# Autodesk Inventor assembly: ASY Beshkino_bio_tank
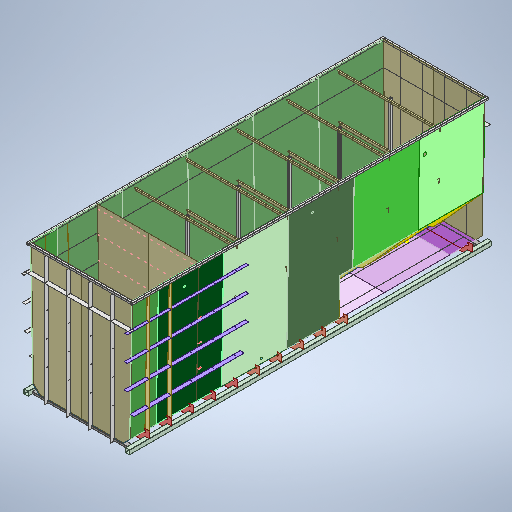
[picture p0: Inventor's stored thumbnail of the model, 512x512]
Saved by Autodesk Inventor 2025 (Build 290162010, 162A)
## iProperties
Created: 2024-07-21
Part Number: ASY Beshkino_bio_tank
Document SubType Name: Assembly
Designer: admin
Mass: 5.81287e+06 g
Surface Area: 2.77755e+06 cm^2
Volume: 3.12018e+06 cm^3
Density: 1.86299 g/cm^3
Author: admin
## Documents named in this file (39)
- C:\Users\pokla\Documents\Inventor\BSH_Beshkino_bio_tank\ASY Beshkino_bio_tank.iam
- C:\Users\pokla\Documents\Inventor\BSH_Beshkino_bio_tank\BSH 000 dim Beshkino_bio_tank.ipt
- C:\Users\pokla\Documents\Inventor\BSH_Beshkino_bio_tank\BSH 010 floor 1.ipt
- C:\Users\pokla\Documents\Inventor\BSH_Beshkino_bio_tank\BSH 021 rib 1.ipt
- C:\Users\pokla\Documents\Inventor\BSH_Beshkino_bio_tank\BSH 022 rib 2.ipt
- C:\Users\pokla\Documents\Inventor\BSH_Beshkino_bio_tank\BSH 061 tube 1.ipt
- C:\Users\pokla\Documents\Inventor\BSH_Beshkino_bio_tank\BSH 031 nose 1.ipt
- C:\Users\pokla\Documents\Inventor\BSH_Beshkino_bio_tank\BSH 032 board 2.ipt
- C:\Users\pokla\Documents\Inventor\BSH_Beshkino_bio_tank\BSH 033 board 3.ipt
- C:\Users\pokla\Documents\Inventor\BSH_Beshkino_bio_tank\BSH 041 stringer 1.ipt
- C:\Users\pokla\Documents\Inventor\BSH_Beshkino_bio_tank\BSH 039 back 9.ipt
- C:\Users\pokla\Documents\Inventor\BSH_Beshkino_bio_tank\BSH 041 stringer floor.ipt
- C:\Users\pokla\Documents\Inventor\BSH_Beshkino_bio_tank\BSH 062 tube 2.ipt
- C:\Users\pokla\Documents\Inventor\BSH_Beshkino_bio_tank\BSH 042 stringer 2.ipt
- C:\Users\pokla\Documents\Inventor\BSH_Beshkino_bio_tank\BSH 043 stringer 3.ipt
- C:\Users\pokla\Documents\Inventor\BSH_Beshkino_bio_tank\BSH 044 stringer 4.ipt
- C:\Users\pokla\Documents\Inventor\BSH_Beshkino_bio_tank\BSH 042 stringer floor.ipt
- C:\Users\pokla\Documents\Inventor\BSH_Beshkino_bio_tank\BSH 045 stringer 1.ipt
- C:\Users\pokla\Documents\Inventor\BSH_Beshkino_bio_tank\BSH 045 stringer 5.ipt
- C:\Users\pokla\Documents\Inventor\BSH_Beshkino_bio_tank\BSH 033 board cone 3.ipt
- C:\Users\pokla\Documents\Inventor\BSH_Beshkino_bio_tank\BSH 034 board cone 4.ipt
- C:\Users\pokla\Documents\Inventor\BSH_Beshkino_bio_tank\BSH 035 divider 1.ipt
- C:\Users\pokla\Documents\Inventor\BSH_Beshkino_bio_tank\BSH 036 divider 2.ipt
- C:\Users\pokla\Documents\Inventor\BSH_Beshkino_bio_tank\BSH 012 floor 2.ipt
- C:\Users\pokla\Documents\Inventor\BSH_Beshkino_bio_tank\BSH 037 cone 3.ipt
- C:\Users\pokla\Documents\Inventor\BSH_Beshkino_bio_tank\BSH 013 floor 3.ipt
- C:\Users\pokla\Documents\Inventor\BSH_Beshkino_bio_tank\BSH 015 board cone 5.ipt
- C:\Users\pokla\Documents\Inventor\BSH_Beshkino_bio_tank\BSH 038 divider.ipt
- C:\Users\pokla\Documents\Inventor\BSH_Beshkino_bio_tank\BSH 046 stringer 6.ipt
- C:\Users\pokla\Documents\Inventor\BSH_Beshkino_bio_tank\BSH 035 board cone 5.ipt
- C:\Users\pokla\Documents\Inventor\BSH_Beshkino_bio_tank\BSH 035 board .ipt
- C:\Users\pokla\Documents\Inventor\BSH_Beshkino_bio_tank\BSH 051 back 1.ipt
- C:\Users\pokla\Documents\Inventor\BSH_Beshkino_bio_tank\BSH 052 board 2.ipt
- C:\Users\pokla\Documents\Inventor\BSH_Beshkino_bio_tank\BSH 053 board 3.ipt
- C:\Users\pokla\Documents\Inventor\BSH_Beshkino_bio_tank\BSH 054 board cone 4.ipt
- C:\Users\pokla\Documents\Inventor\BSH_Beshkino_bio_tank\BSH 063 tube 3.ipt
- C:\Users\pokla\Documents\Inventor\BSH_Beshkino_bio_tank\BSH 064 tube 4.ipt
- C:\Users\pokla\Documents\Inventor\BSH_Beshkino_bio_tank\BSH 065 tube 5.ipt
- C:\Users\pokla\Documents\Inventor\BSH_Beshkino_bio_tank\BSH 023 rib 3.ipt
## Components (116 placed, 43 different names)
1. BSH 000 dim Beshkino_bio_tank.ipt:1
2. BSH 022 rib 2.ipt:1 — Rigid:27, Rigid:28, Rigid:29, Rigid:30, Rigid:74, Mate:104, Flush:26
3. BSH 061 tube 1.ipt:1 — Mate:1, Rigid:1, Mate:3, Flush:12, Mate:66, Mate:67, Mate:95, Flush:23
4. BSH 061 tube 1.ipt:2 — Mate:2, Rigid:1, Mate:4, Flush:3, Flush:4, Flush:16, Mate:65, Flush:20
5. BSH 062 tube 2.ipt:1 — Mate:19, Flush:12, Flush:16, Mate:65
6. BSH 062 tube 2.ipt:2 — Mate:68, Flush:20, Mate:95, Flush:23
7. BSH 010 floor 1.ipt:2 — Rigid:5, Rigid:83, Mate:77, Flush:18, Flush:19
8. BSH 010 floor 1.ipt:3 — Rigid:5, Rigid:82
9. BSH 010 floor 1.ipt:1 — Mate:5, Mate:6, Mate:7, Flush:4, Mate:10, Flush:5, Flush:11, Flush:17, Mate:70, Rigid:82, Mate:74
10. BSH 031 nose 1.ipt:1 — Mate:10, Flush:5, Mate:11, Rigid:11, Mate:73, Mate:108
11. BSH 033 board 3.ipt:1 — Flush:11, Mate:73, Mate:74, Rigid:104
12. BSH 031 nose 1.ipt:2 — Rigid:11, Rigid:53, Mate:69
13. BSH 021 rib 1.ipt:1 — Mate:4, Flush:3, Mate:5, Mate:6, Rigid:9, Mate:19, Rigid:74, Rigid:76, Rigid:109, Rigid:118, Rigid:122, Rigid:126
14. BSH 045 stringer 1:1
15. BSH 031 nose 1:3 — Mate:113
16. BSH 031 nose 1:4 — Rigid:53, Flush:112
17. BSH 033 board cone 3:1 — Mate:26, Rigid:57, Mate:30, Mate:80, Mate:83
18. BSH 031 nose 1:7 — Mate:26, Mate:30, Mate:84, Flush:21, Mate:94
19. BSH 031 nose 1:8 — Flush:8, Mate:40, Mate:111
20. BSH 033 board cone 3:2 — Rigid:57, Angle:1, Mate:49, Mate:50, Mate:64, Mate:71
21. BSH 043 stringer 3.ipt:1 — Rigid:29
22. BSH 042 stringer 2.ipt:1 — Rigid:28
23. BSH 041 stringer 1.ipt:1 — Rigid:27
24. BSH 041 stringer 1.ipt:2
25. BSH 042 stringer 2.ipt:2
26. BSH 043 stringer 3.ipt:2
27. BSH 044 stringer 4.ipt:2 — Rigid:71, Rigid:127, Mate:109
28. BSH 034 board cone 4:2 — Mate:84, Rigid:108, Mate:88, Mate:89, Mate:90, Mate:91
29. BSH 012 floor 2:1 — Rigid:66, Mate:42, Angle:1, Mate:49, Rigid:83, Mate:72, Mate:87
30. BSH 037 cone 3:1 — Mate:42, Mate:50, Mate:90
31. BSH 033 board 3:2 — Flush:17, Mate:69, Mate:70, Rigid:81
32. BSH 012 floor 2:2 — Rigid:66, Rigid:67, Mate:63, Mate:78, Mate:98
33. BSH 013 floor 3:1 — Rigid:67, Mate:40, Mate:81
34. BSH 039 back 9:2 — Rigid:90, Rigid:103
35. BSH 015 board cone 5:1 — Mate:71, Mate:72, Mate:85, Mate:86
36. BSH 038 divider:1 — Mate:77, Flush:18, Flush:19
37. BSH 046 stringer 6:1 — Mate:107, Mate:108, Mate:109, Rigid:128, Rigid:129, Rigid:130, Rigid:131
38. BSH 037 cone 3:2 — Mate:63, Mate:64, Mate:91
39. BSH 044 stringer 4:3 — Rigid:71, Rigid:72
40. BSH 044 stringer 4:4 — Rigid:72, Mate:112
41. BSH 022 rib 2:34 — Rigid:76, Mate:102, Flush:27, Rigid:127
42. BSH 020 rib 1:4 — Mate:66, Mate:67, Mate:68
43. BSH 022 rib 2:35 — Rigid:77
44. BSH 021 rib 1.ipt:2 — Rigid:9, Rigid:75, Rigid:77
45. BSH 037 cone 3:3 — Mate:78, Mate:80, Mate:88
46. BSH 037 cone 3:4 — Mate:81, Mate:83, Mate:89
47. BSH 035 board cone 5:1 — Rigid:107
48. BSH 035 board :1 — Rigid:90, Mate:85, Rigid:106
49. BSH 020 rib 1:5
50. BSH 020 rib 1:6
51. BSH 020 rib 1:7 — Rigid:94
52. BSH 020 rib 1:8 — Rigid:94
53. BSH 020 rib 1:9
54. BSH 020 rib 1:10
55. BSH 020 rib 1:11
56. BSH 051 back 1:1 — Rigid:103, Flush:21, Mate:96
57. BSH 052 board 2:1 — Rigid:104, Rigid:105
58. BSH 044 stringer 4.ipt:1 — Rigid:30
59. BSH 022 rib 2:33 — Rigid:75
60. BSH 053 board 3:1 — Rigid:105, Rigid:106
61. BSH 054 board cone 4:1 — Rigid:107, Rigid:108, Mate:86, Mate:87
62. BSH 041 stringer floor:1 — Rigid:109, Rigid:114
63. BSH 042 stringer floor:1 — Rigid:113
64. BSH 041 stringer floor:2 — Rigid:112, Rigid:114
65. BSH 041 stringer floor:3 — Rigid:112, Rigid:113
66. BSH 020 rib 1:12
67. BSH 041 stringer floor:4 — Rigid:118
68. BSH 042 stringer floor:2
69. BSH 041 stringer floor:5
70. BSH 041 stringer floor:6
71. BSH 041 stringer floor:7 — Rigid:122
72. BSH 042 stringer floor:3
73. BSH 041 stringer floor:8
74. BSH 041 stringer floor:9
75. BSH 041 stringer floor:10 — Rigid:126
76. BSH 042 stringer floor:4
77. BSH 041 stringer floor:11
78. BSH 041 stringer floor:12
79. BSH 064 tube 4:1 — Mate:100, Mate:102, Flush:27, Flush:28, Flush:29, Flush:30, Flush:31
80. BSH 064 tube 4:2 — Mate:103, Mate:104, Flush:26
81. BSH 065 tube 5:1 — Mate:105, Flush:28, Flush:29
82. BSH 065 tube 5:2 — Mate:106, Flush:30, Flush:31
83. BSH 023 rib 3:1 — Rigid:128
84. BSH 023 rib 3:2 — Rigid:129
85. BSH 023 rib 3:3 — Rigid:130
86. BSH 023 rib 3:4 — Rigid:131
87. BSH 046 stringer 6:2 — Flush:111, Mate:111, Mate:112
88. BSH 023 rib 3:5
89. BSH 023 rib 3:6
90. BSH 023 rib 3:7
91. BSH 023 rib 3:8
92. BSH 032 board 2:4 — Rigid:81
93. BSH 032 board 2:5
94. BSH 032 board 2:6
95. BSH 032 board 2:7
96. BSH 032 board 2:8
97. BSH 035 divider 1:1 — Flush:22, Mate:94, Mate:96, Flush:24, Mate:97
98. BSH 036 divider 2:1 — Flush:22, Mate:93, Flush:24, Mate:99
99. BSH 063 tube 3:1 — Mate:98, Mate:99, Flush:25
100. BSH 035 divider 1:2
101. BSH 036 divider 2:2
102. BSH 063 tube 3:2
103. BSH 035 divider 1:3
104. BSH 036 divider 2:3
105. BSH 063 tube 3:3
106. BSH 035 divider 1:4
107. BSH 036 divider 2:4
108. BSH 063 tube 3:4
109. BSH 035 divider 1:5
110. BSH 036 divider 2:5
111. BSH 063 tube 3:5
112. BSH 045 stringer 5:1 — Mate:23, Flush:112, Mate:113
113. BSH 045 stringer 5:2
114. BSH 045 stringer 5:3
115. BSH 045 stringer 5:4
116. BSH 045 stringer 5:5
## Component patterns: (5 elements, first: BSH 032 board 2:4), (5 elements, first: BSH 035 divider 1:1 + BSH 036 divider 2:1 + BSH 063 tube 3:1), (5 elements, first: BSH 045 stringer 5:1)
## Relationships (142: Mate 61, WeldJoint 56, Flush 24, Angle 1)
- Mate:1: BSH 061 tube 1.ipt:1
- Mate:2: BSH 061 tube 1.ipt:2
- Rigid:1 [WeldJoint] (-2400 mm): BSH 061 tube 1.ipt:1 ↔ BSH 061 tube 1.ipt:2
- Mate:3: BSH 061 tube 1.ipt:1
- Mate:4: BSH 061 tube 1.ipt:2 ↔ BSH 021 rib 1.ipt:1
- Flush:3: BSH 061 tube 1.ipt:2 ↔ BSH 021 rib 1.ipt:1
- Mate:5: BSH 010 floor 1.ipt:1 ↔ BSH 021 rib 1.ipt:1
- Mate:6: BSH 010 floor 1.ipt:1 ↔ BSH 021 rib 1.ipt:1
- Rigid:5 [WeldJoint]: BSH 010 floor 1.ipt:2 ↔ BSH 010 floor 1.ipt:3
- Mate:7: BSH 010 floor 1.ipt:1
- Flush:4 (100 mm): BSH 061 tube 1.ipt:2 ↔ BSH 010 floor 1.ipt:1
- Rigid:9 [WeldJoint] (-500 mm): BSH 021 rib 1.ipt:1 ↔ BSH 021 rib 1.ipt:2
- Mate:10: BSH 010 floor 1.ipt:1 ↔ BSH 031 nose 1.ipt:1
- Flush:5 (10 mm): BSH 010 floor 1.ipt:1 ↔ BSH 031 nose 1.ipt:1
- Mate:11: BSH 031 nose 1.ipt:1
- Rigid:11 [WeldJoint]: BSH 031 nose 1.ipt:1 ↔ BSH 031 nose 1.ipt:2
- Rigid:27 [WeldJoint] (2 mm): BSH 022 rib 2.ipt:1 ↔ BSH 041 stringer 1.ipt:1
- Rigid:28 [WeldJoint] (2 mm): BSH 022 rib 2.ipt:1 ↔ BSH 042 stringer 2.ipt:1
- Rigid:29 [WeldJoint] (2 mm): BSH 022 rib 2.ipt:1 ↔ BSH 043 stringer 3.ipt:1
- Rigid:30 [WeldJoint] (2 mm): BSH 022 rib 2.ipt:1 ↔ BSH 044 stringer 4.ipt:1
- Mate:19 (248.5 mm): BSH 062 tube 2.ipt:1 ↔ BSH 021 rib 1.ipt:1
- Mate:23: BSH 045 stringer 5:1
- [WeldJoint]: BSH 031 nose 1:3 ↔ BSH 031 nose 1:4
- Rigid:53 [WeldJoint] (1500 mm): BSH 031 nose 1.ipt:2 ↔ BSH 031 nose 1:4
- [WeldJoint]: BSH 031 nose 1:7 ↔ BSH 031 nose 1:8
- Flush:8: BSH 031 nose 1:8
- Mate:26: BSH 033 board cone 3:1 ↔ BSH 031 nose 1:7
- Rigid:57 [WeldJoint]: BSH 033 board cone 3:1 ↔ BSH 033 board cone 3:2
- Mate:30: BSH 033 board cone 3:1 ↔ BSH 031 nose 1:7
- Flush:11: BSH 010 floor 1.ipt:1 ↔ BSH 033 board 3.ipt:1
- Rigid:66 [WeldJoint]: BSH 012 floor 2:1 ↔ BSH 012 floor 2:2
- Rigid:67 [WeldJoint]: BSH 012 floor 2:2 ↔ BSH 013 floor 3:1
- Mate:40: BSH 031 nose 1:8 ↔ BSH 013 floor 3:1
- Mate:42: BSH 012 floor 2:1 ↔ BSH 037 cone 3:1
- Angle:1 (132 deg): BSH 033 board cone 3:2 ↔ BSH 012 floor 2:1
- Mate:49: BSH 033 board cone 3:2 ↔ BSH 012 floor 2:1
- Mate:50: BSH 033 board cone 3:2 ↔ BSH 037 cone 3:1
- Flush:12: BSH 061 tube 1.ipt:1 ↔ BSH 062 tube 2.ipt:1
- Mate:63: BSH 012 floor 2:2 ↔ BSH 037 cone 3:2
- Mate:64: BSH 033 board cone 3:2 ↔ BSH 037 cone 3:2
- Rigid:71 [WeldJoint] (-10 mm): BSH 044 stringer 4.ipt:2 ↔ BSH 044 stringer 4:3
- Rigid:72 [WeldJoint] (-10 mm): BSH 044 stringer 4:3 ↔ BSH 044 stringer 4:4
- Rigid:74 [WeldJoint] (-10 mm): BSH 022 rib 2.ipt:1 ↔ BSH 021 rib 1.ipt:1
- Flush:16 (90 mm): BSH 061 tube 1.ipt:2 ↔ BSH 062 tube 2.ipt:1
- Mate:65: BSH 061 tube 1.ipt:2 ↔ BSH 062 tube 2.ipt:1
- Rigid:75 [WeldJoint] (-10 mm): BSH 021 rib 1.ipt:2 ↔ BSH 022 rib 2:33
- Rigid:76 [WeldJoint] (-10 mm): BSH 021 rib 1.ipt:1 ↔ BSH 022 rib 2:34
- Rigid:77 [WeldJoint] (-10 mm): BSH 022 rib 2:35 ↔ BSH 021 rib 1.ipt:2
- Mate:66: BSH 061 tube 1.ipt:1 ↔ BSH 020 rib 1:4
- Mate:67: BSH 061 tube 1.ipt:1 ↔ BSH 020 rib 1:4
- Mate:68 (248.5 mm): BSH 062 tube 2.ipt:2 ↔ BSH 020 rib 1:4
- Flush:17: BSH 010 floor 1.ipt:1 ↔ BSH 033 board 3:2
- Mate:69: BSH 031 nose 1.ipt:2 ↔ BSH 033 board 3:2
- Mate:70: BSH 010 floor 1.ipt:1 ↔ BSH 033 board 3:2
- Rigid:81 [WeldJoint]: BSH 033 board 3:2 ↔ BSH 032 board 2:4
- Rigid:82 [WeldJoint]: BSH 010 floor 1.ipt:3 ↔ BSH 010 floor 1.ipt:1
- Rigid:83 [WeldJoint]: BSH 010 floor 1.ipt:2 ↔ BSH 012 floor 2:1
- Mate:71: BSH 033 board cone 3:2 ↔ BSH 015 board cone 5:1
- Mate:72: BSH 012 floor 2:1 ↔ BSH 015 board cone 5:1
- Mate:73: BSH 031 nose 1.ipt:1 ↔ BSH 033 board 3.ipt:1
- Mate:74: BSH 010 floor 1.ipt:1 ↔ BSH 033 board 3.ipt:1
- Mate:77: BSH 010 floor 1.ipt:2 ↔ BSH 038 divider:1
- Flush:18: BSH 010 floor 1.ipt:2 ↔ BSH 038 divider:1
- Flush:19: BSH 010 floor 1.ipt:2 ↔ BSH 038 divider:1
- Mate:78: BSH 012 floor 2:2 ↔ BSH 037 cone 3:3
- Mate:80: BSH 033 board cone 3:1 ↔ BSH 037 cone 3:3
- Mate:81: BSH 013 floor 3:1 ↔ BSH 037 cone 3:4
- Mate:83: BSH 033 board cone 3:1 ↔ BSH 037 cone 3:4
- Mate:84: BSH 031 nose 1:7 ↔ BSH 034 board cone 4:2
- Rigid:90 [WeldJoint]: BSH 039 back 9:2 ↔ BSH 035 board :1
- Mate:85: BSH 015 board cone 5:1 ↔ BSH 035 board :1
- Rigid:94 [WeldJoint] (500 mm): BSH 020 rib 1:7 ↔ BSH 020 rib 1:8
- Flush:20: BSH 061 tube 1.ipt:2 ↔ BSH 062 tube 2.ipt:2
- Rigid:103 [WeldJoint]: BSH 039 back 9:2 ↔ BSH 051 back 1:1
- Rigid:104 [WeldJoint]: BSH 033 board 3.ipt:1 ↔ BSH 052 board 2:1
- Rigid:105 [WeldJoint]: BSH 052 board 2:1 ↔ BSH 053 board 3:1
- Rigid:106 [WeldJoint]: BSH 035 board :1 ↔ BSH 053 board 3:1
- Flush:21 (10 mm): BSH 031 nose 1:7 ↔ BSH 051 back 1:1
- Rigid:107 [WeldJoint]: BSH 035 board cone 5:1 ↔ BSH 054 board cone 4:1
- Rigid:108 [WeldJoint]: BSH 034 board cone 4:2 ↔ BSH 054 board cone 4:1
- Mate:86: BSH 015 board cone 5:1 ↔ BSH 054 board cone 4:1
- Mate:87: BSH 012 floor 2:1 ↔ BSH 054 board cone 4:1
- Mate:88: BSH 034 board cone 4:2 ↔ BSH 037 cone 3:3
- Mate:89: BSH 034 board cone 4:2 ↔ BSH 037 cone 3:4
- Mate:90: BSH 034 board cone 4:2 ↔ BSH 037 cone 3:1
- Mate:91: BSH 034 board cone 4:2 ↔ BSH 037 cone 3:2
- Flush:22: BSH 035 divider 1:1 ↔ BSH 036 divider 2:1
- Mate:93: BSH 036 divider 2:1
- Mate:94 (1000 mm): BSH 031 nose 1:7 ↔ BSH 035 divider 1:1
- Rigid:109 [WeldJoint] (2 mm): BSH 021 rib 1.ipt:1 ↔ BSH 041 stringer floor:1
- Mate:95: BSH 061 tube 1.ipt:1 ↔ BSH 062 tube 2.ipt:2
- Flush:23 (90 mm): BSH 061 tube 1.ipt:1 ↔ BSH 062 tube 2.ipt:2
- Rigid:112 [WeldJoint] (-20 mm): BSH 041 stringer floor:2 ↔ BSH 041 stringer floor:3
- Rigid:113 [WeldJoint] (-250.2 mm): BSH 042 stringer floor:1 ↔ BSH 041 stringer floor:3
- Rigid:114 [WeldJoint] (-20 mm): BSH 041 stringer floor:1 ↔ BSH 041 stringer floor:2
- [WeldJoint] (-20 mm): BSH 041 stringer floor:5 ↔ BSH 041 stringer floor:6
- [WeldJoint] (-250.2 mm): BSH 042 stringer floor:2 ↔ BSH 041 stringer floor:6
- [WeldJoint] (-20 mm): BSH 041 stringer floor:4 ↔ BSH 041 stringer floor:5
- Rigid:118 [WeldJoint] (2 mm): BSH 021 rib 1.ipt:1 ↔ BSH 041 stringer floor:4
- [WeldJoint] (-20 mm): BSH 041 stringer floor:8 ↔ BSH 041 stringer floor:9
- [WeldJoint] (-250.2 mm): BSH 042 stringer floor:3 ↔ BSH 041 stringer floor:9
- [WeldJoint] (-20 mm): BSH 041 stringer floor:7 ↔ BSH 041 stringer floor:8
- Rigid:122 [WeldJoint] (2 mm): BSH 021 rib 1.ipt:1 ↔ BSH 041 stringer floor:7
- [WeldJoint] (-20 mm): BSH 041 stringer floor:11 ↔ BSH 041 stringer floor:12
- [WeldJoint] (-250.2 mm): BSH 042 stringer floor:4 ↔ BSH 041 stringer floor:12
- [WeldJoint] (-20 mm): BSH 041 stringer floor:10 ↔ BSH 041 stringer floor:11
- Rigid:126 [WeldJoint] (2 mm): BSH 021 rib 1.ipt:1 ↔ BSH 041 stringer floor:10
- Mate:96 (100 mm): BSH 051 back 1:1 ↔ BSH 035 divider 1:1
- Flush:24 (1000 mm): BSH 035 divider 1:1 ↔ BSH 036 divider 2:1
- Mate:97: BSH 035 divider 1:1
- Mate:98: BSH 012 floor 2:2 ↔ BSH 063 tube 3:1
- Mate:99: BSH 036 divider 2:1 ↔ BSH 063 tube 3:1
- Flush:25: BSH 063 tube 3:1
- Mate:100: BSH 064 tube 4:1
- Mate:102: BSH 022 rib 2:34 ↔ BSH 064 tube 4:1
- Mate:103: BSH 064 tube 4:2
- Mate:104: BSH 022 rib 2.ipt:1 ↔ BSH 064 tube 4:2
- Flush:26: BSH 022 rib 2.ipt:1 ↔ BSH 064 tube 4:2
- Flush:27: BSH 022 rib 2:34 ↔ BSH 064 tube 4:1
- Mate:105: BSH 065 tube 5:1
- Flush:28: BSH 064 tube 4:1 ↔ BSH 065 tube 5:1
- Flush:29: BSH 064 tube 4:1 ↔ BSH 065 tube 5:1
- Mate:106: BSH 065 tube 5:2
- Flush:30: BSH 064 tube 4:1 ↔ BSH 065 tube 5:2
- Flush:31: BSH 064 tube 4:1 ↔ BSH 065 tube 5:2
- Rigid:127 [WeldJoint] (2 mm): BSH 044 stringer 4.ipt:2 ↔ BSH 022 rib 2:34
- Mate:107: BSH 046 stringer 6:1
- Mate:108: BSH 031 nose 1.ipt:1 ↔ BSH 046 stringer 6:1
- Mate:109: BSH 044 stringer 4.ipt:2 ↔ BSH 046 stringer 6:1
- Rigid:128 [WeldJoint] (2 mm): BSH 046 stringer 6:1 ↔ BSH 023 rib 3:1
- Rigid:129 [WeldJoint] (2 mm): BSH 046 stringer 6:1 ↔ BSH 023 rib 3:2
- Rigid:130 [WeldJoint] (2 mm): BSH 046 stringer 6:1 ↔ BSH 023 rib 3:3
- Rigid:131 [WeldJoint] (2 mm): BSH 046 stringer 6:1 ↔ BSH 023 rib 3:4
- [WeldJoint] (2 mm): BSH 046 stringer 6:2 ↔ BSH 023 rib 3:5
- [WeldJoint] (2 mm): BSH 046 stringer 6:2 ↔ BSH 023 rib 3:6
- [WeldJoint] (2 mm): BSH 046 stringer 6:2 ↔ BSH 023 rib 3:7
- [WeldJoint] (2 mm): BSH 046 stringer 6:2 ↔ BSH 023 rib 3:8
- Flush:111: BSH 046 stringer 6:2
- Mate:111: BSH 031 nose 1:8 ↔ BSH 046 stringer 6:2
- Mate:112: BSH 044 stringer 4:4 ↔ BSH 046 stringer 6:2
- Flush:112 (100 mm): BSH 031 nose 1:4 ↔ BSH 045 stringer 5:1
- Mate:113: BSH 031 nose 1:3 ↔ BSH 045 stringer 5:1
## Named parameters: d118_d31 = 0 mm, d124_d31 = 0 mm, d324_d323 = -20 mm, d325_d318 = -20 mm, d326_d319 = -250.2 mm, d328_d323 = -20 mm, d329_d318 = -20 mm, d330_d319 = -250.2 mm, d332_d323 = -20 mm, d333_d318 = -20 mm, d334_d319 = -250.2 mm, d381_d380 = 2 mm, d382_d377 = 2 mm, d383_d378 = 2 mm, d384_d379 = 2 mm
